# Autodesk Inventor assembly: Assembly1_replace
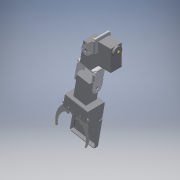
[picture p0: Inventor's stored thumbnail of the model, 180x180]
Saved by Autodesk Inventor 2018 (Build 220112000, 112)
## iProperties
Created: 2018-09-29
Part Number: Assembly1_replace
Document SubType Name: Assembly
Designer: Abhay
Author: Abhay
## Documents named in this file (6)
- C:\Users\Abhay\Desktop\Huro\gripper\Assembly1_replace.iam
- C:\Users\Abhay\Desktop\Huro\gripper\Solid1_12.ipt
- C:\Users\Abhay\Desktop\Huro\gripper\Spur Gears1.iam
- C:\Users\Abhay\Desktop\Huro\gripper\ax_18_replace.ipt
- C:\Users\Abhay\Desktop\Huro\gripper\Solid1_9.ipt
- C:\Users\Abhay\Desktop\Huro\gripper\Solid1_8.ipt
## Components (8 placed, 5 different names)
1. Part34:1 — Rotational:1, Mate:1, Rotational:3
2. Spur Gears:12 [sub-assembly] — Rotational:1, Mate:1, Rotational:2
3. ax_18_replace:3 — Rotational:2
4. ax_18_replace:4 — Rotational:3, Rotational:4
5. ax_18_replace:5 — Mate:2, Rotational:5
6. Solid1_9:1 — Rotational:4, Mate:2
7. Solid1_8:1 — Rotational:5, Rotational:6
8. ax_18_replace:6 — Rotational:6, Mate:3, Mate:4
## Relationships (11: RevoluteJoint 6, Mate 5)
- Rotational:1 [RevoluteJoint]: Part34:1 ↔ Spur Gears:12
- Mate:1: Part34:1 ↔ Spur Gears:12
- Rotational:2 [RevoluteJoint]: Spur Gears:12 ↔ ax_18_replace:3
- Rotational:3 [RevoluteJoint]: Part34:1 ↔ ax_18_replace:4
- Rotational:4 [RevoluteJoint]: ax_18_replace:4 ↔ Solid1_9:1
- Mate:2: ax_18_replace:5 ↔ Solid1_9:1
- Rotational:5 [RevoluteJoint]: ax_18_replace:5 ↔ Solid1_8:1
- Rotational:6 [RevoluteJoint]: Solid1_8:1 ↔ ax_18_replace:6
- Mate:3: ax_18_replace:6
- Mate:4: ax_18_replace:6
- Mate:5
